# Autodesk Inventor assembly: Wheel Original
Saved by Autodesk Inventor 2014 SP1 (Build 180222100, 222)
## iProperties
Created: 2014-01-12
Part Number: Wheel Original
Document SubType Name: Assembly
Designer: tom
Author: tom
## Documents named in this file (3)
- C:\Users\tom\Documents\GitHub\Vacubot\Inventor\Wheel Original.iam
- C:\Users\tom\Documents\GitHub\Vacubot\Inventor\Wheel Bar.ipt
- C:\Users\tom\Documents\GitHub\Vacubot\Inventor\Front Wheel.ipt
## Components (2 placed, 2 different names)
1. Wheel Bar:1
2. Front Wheel:1
## Relationships (1: RevoluteJoint 1)
- [RevoluteJoint]: Wheel Bar:1 ↔ Front Wheel:1
